# Autodesk Inventor assembly: Cockpit
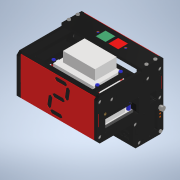
[picture p0: Inventor's stored thumbnail of the model, 180x180]
Saved by Autodesk Inventor 2020 (Build 240168000, 168)
## iProperties
Created: 2022-04-24
Part Number: Cockpit
Document SubType Name: Assembly
Designer: Masato Kubotera
Author: Masato Kubotera
## Documents named in this file (33)
- C:\Users\MasatoKubotera\Documents\Inventor\SUSTAINA-OP\UpperBody\Cockpit\Cockpit.iam
- C:\Users\MasatoKubotera\Documents\Inventor\SUSTAINA-OP\UpperBody\Cockpit\Cockpit_side_frame_MIR.ipt
- C:\Users\MasatoKubotera\Documents\Inventor\SUSTAINA-OP\UpperBody\Cockpit\Cockpit_battery_bottom_frame.ipt
- C:\Users\MasatoKubotera\Documents\Inventor\SUSTAINA-OP\UpperBody\Cockpit\Cockpit_battery_front_frame.ipt
- C:\Users\MasatoKubotera\Documents\Inventor\SUSTAINA-OP\UpperBody\Cockpit\Cockpit_front_frame.ipt
- C:\Users\MasatoKubotera\Documents\Inventor\SUSTAINA-OP\UpperBody\Cockpit\Cockpit_carrier_board_frame.ipt
- C:\Users\MasatoKubotera\Documents\Inventor\SUSTAINA-OP\UpperBody\Cockpit\Cockpit_back_frame.ipt
- C:\Users\MasatoKubotera\Documents\Inventor\SUSTAINA-OP\UpperBody\Cockpit\Cockpit_circuit_board_frame.ipt
- C:\Users\MasatoKubotera\Documents\Inventor\SUSTAINA-OP\UpperBody\Cockpit\Cockpit_battery_back_door.ipt
- C:\Users\MasatoKubotera\Documents\Inventor\SUSTAINA-OP\UpperBody\Cockpit\Cockpit_side_frame.ipt
- C:\Users\MasatoKubotera\Documents\Inventor\SUSTAINA-OP\ReadyMade\InsertNut\IRU-304S.ipt
- C:\Users\MasatoKubotera\Documents\Inventor\SUSTAINA-OP\ReadyMade\InsertNut\UD-43040.ipt
- C:\Users\MasatoKubotera\Documents\Inventor\SUSTAINA-OP\ReadyMade\Neodymium_magnet_Phi3_T3.ipt
- C:\Users\MasatoKubotera\Documents\Inventor\SUSTAINA-OP\UpperBody\Cockpit\Cockpit_front_frame_cloth.ipt
- C:\Users\MasatoKubotera\Documents\Inventor\SUSTAINA-OP\UpperBody\Cockpit\Cockpit_back_frame_cloth.ipt
- C:\Users\MasatoKubotera\Documents\Inventor\SUSTAINA-OP\ReadyMade\JetsonXavierNX_and_EN715.ipt
- C:\Users\MasatoKubotera\Documents\Inventor\SUSTAINA-OP\UpperBody\Cockpit\MainBoard.ipt
- C:\Users\MasatoKubotera\Documents\Inventor\SUSTAINA-OP\UpperBody\Cockpit\MainBoard_cover.ipt
- C:\Users\MasatoKubotera\Documents\Inventor\SUSTAINA-OP\ReadyMade\Battery\HP-G830C2800S3.ipt
- C:\Users\MasatoKubotera\Documents\Inventor\SUSTAINA-OP\ReadyMade\Screw\M3-6.ipt
- C:\Users\MasatoKubotera\Documents\Inventor\SUSTAINA-OP\ReadyMade\Screw\M3-10.ipt
- C:\Users\MasatoKubotera\Documents\Inventor\SUSTAINA-OP\ReadyMade\Screw\M3-8.ipt
- C:\Users\MasatoKubotera\Documents\Inventor\SUSTAINA-OP\UpperBody\Cockpit\Cockpit_top_frame.ipt
- C:\Users\MasatoKubotera\Documents\Inventor\SUSTAINA-OP\UpperBody\Cockpit\StartStopSwitch.ipt
- C:\Users\MasatoKubotera\Documents\Inventor\SUSTAINA-OP\ReadyMade\Spacer\ASL-313BE.ipt
- C:\Users\MasatoKubotera\Documents\Inventor\SUSTAINA-OP\ReadyMade\Spacer\BSL-306.5BE.ipt
- C:\Users\MasatoKubotera\Documents\Inventor\SUSTAINA-OP\UpperBody\Cockpit\ExpansionBoard.ipt
- C:\Users\MasatoKubotera\Documents\Inventor\SUSTAINA-OP\ReadyMade\Screw\M2_6-10.ipt
- C:\Users\MasatoKubotera\Documents\Inventor\SUSTAINA-OP\ReadyMade\Screw\SPNFL-BRN-M3-10.ipt
- C:\Users\MasatoKubotera\Documents\Inventor\SUSTAINA-OP\UpperBody\Cockpit\MainBoard_fan_plate.ipt
- C:\Users\MasatoKubotera\Documents\Inventor\SUSTAINA-OP\ReadyMade\YDM2507C12F.ipt
- C:\Users\MasatoKubotera\Documents\Inventor\SUSTAINA-OP\ReadyMade\Spacer\BRU-309S.ipt
- C:\Users\MasatoKubotera\Documents\Inventor\SUSTAINA-OP\ReadyMade\Screw\M2-6.ipt
## Components (121 placed, 32 different names)
1. MainBoard:1 — 挿入:63, 挿入:64, 挿入:65, 挿入:66, 挿入:95, 挿入:96, 挿入:148, 挿入:149
2. StartStopSwitch:1 — 挿入:103, 挿入:104, 挿入:105, 挿入:106
3. ExpansionBoard:1 — 挿入:123, 挿入:124, 挿入:125, 挿入:126, 挿入:127, 挿入:128, 挿入:129, 挿入:130
4. JetsonXavierNX_and_EN715:1 — 挿入:115, 挿入:116, 挿入:117, 挿入:118, 挿入:119, 挿入:120, 挿入:121, 挿入:122
5. M2-6:1 — 挿入:153
6. M2-6:2 — 挿入:152
7. Cockpit_side_frame_MIR:1 — 挿入:11, 挿入:12, 挿入:23, 挿入:24, 挿入:27, 挿入:28, 挿入:31, 挿入:32, 挿入:35, 挿入:36, 挿入:38, 挿入:40, 挿入:42, 挿入:46, 挿入:47, 挿入:48, 挿入:75, 挿入:77, 挿入:78, 挿入:79, 挿入:80, 挿入:81, 挿入:82, 挿入:134, 挿入:137
8. Cockpit_battery_bottom_frame:1 — 挿入:17, 挿入:18, 角度:2
9. Cockpit_battery_front_frame:1 — 挿入:19, 挿入:20, 角度:1
10. Cockpit_front_frame:1 — 挿入:1, 挿入:2, 挿入:3, フラッシュ:4, メイト:1
11. Cockpit_carrier_board_frame:1 — 挿入:5, 挿入:6, 挿入:7, 挿入:8, 挿入:89, 挿入:90, 挿入:91, 挿入:92, 挿入:111, 挿入:112, 挿入:113, 挿入:114
12. Cockpit_back_frame:1 — 挿入:13, 挿入:14, 挿入:15, 挿入:16, フラッシュ:7, メイト:2, 挿入:131, 挿入:132, 挿入:152, 挿入:153
13. Cockpit_circuit_board_frame:1 — メイト:3, メイト:4, フラッシュ:8, 挿入:55, 挿入:56, 挿入:57, 挿入:58
14. Cockpit_battery_back_door:1 — 挿入:41, 挿入:42, 挿入:49, 挿入:50, 挿入:51, 挿入:52, 挿入:53, 挿入:54, 角度:3
15. Cockpit_side_frame:1 — フラッシュ:1, フラッシュ:2, フラッシュ:3, 挿入:9, 挿入:10, 挿入:21, 挿入:22, 挿入:25, 挿入:26, 挿入:29, 挿入:30, 挿入:33, 挿入:34, 挿入:37, 挿入:39, 角度:1, 角度:2, 挿入:41, 挿入:43, 挿入:44, 挿入:45, フラッシュ:6, メイト:3, メイト:4, フラッシュ:8, 挿入:67, 挿入:68, 挿入:69, 挿入:70, 挿入:71, 挿入:72, 挿入:73, 挿入:74, 挿入:133, 角度:3, フラッシュ:5
16. Cockpit_front_frame_cloth:1 — フラッシュ:4, フラッシュ:5, メイト:1
17. Cockpit_back_frame_cloth:1 — フラッシュ:6, フラッシュ:7, メイト:2
18. Cockpit_top_frame:1 — 挿入:97, 挿入:98, 挿入:99, 挿入:100, 挿入:101, 挿入:102, 挿入:107, 挿入:108, 挿入:109, 挿入:110
19. MainBoard_cover:1 — 挿入:59, 挿入:60, 挿入:61, 挿入:62, 挿入:63, 挿入:64, 挿入:65, 挿入:66
20. MainBoard_fan_plate:1 — 挿入:138, 挿入:139, 挿入:140, 挿入:141, 挿入:146, 挿入:147, 挿入:150, 挿入:151
21. UD-43040:1 — 挿入:21
22. UD-43040:2 — 挿入:22, 挿入:83
23. UD-43040:3 — 挿入:23
24. UD-43040:4 — 挿入:24, 挿入:84
25. UD-43040:5 — 挿入:55, 挿入:59
26. UD-43040:6 — 挿入:56, 挿入:60
27. UD-43040:7 — 挿入:57, 挿入:61
28. UD-43040:8 — 挿入:58, 挿入:62
29. UD-43040:9 — 挿入:101, 挿入:103
30. UD-43040:10 — 挿入:102, 挿入:104
31. UD-43040:11 — 挿入:133, 挿入:135
32. UD-43040:12 — 挿入:134, 挿入:136
33. HP-G830C2800S3:1
34. ASL-313BE:1 — 挿入:115, 挿入:123
35. ASL-313BE:2 — 挿入:116, 挿入:124
36. ASL-313BE:3 — 挿入:117, 挿入:126
37. ASL-313BE:4 — 挿入:118, 挿入:125
38. BSL-306.5BE:1 — 挿入:111, 挿入:119
39. BSL-306.5BE:2 — 挿入:112, 挿入:120
40. BSL-306.5BE:3 — 挿入:113, 挿入:122
41. BSL-306.5BE:4 — 挿入:114, 挿入:121
42. BRU-309S:2 — 挿入:149, 挿入:151
43. BRU-309S:1 — 挿入:148, 挿入:150
44. IRU-304S:1 — 挿入:1, 挿入:25
45. IRU-304S:2 — 挿入:2, 挿入:26
46. IRU-304S:3 — 挿入:3, 挿入:27
47. IRU-304S:4 — 挿入:28
48. IRU-304S:5 — 挿入:5, 挿入:29
49. IRU-304S:6 — 挿入:6, 挿入:30
50. IRU-304S:7 — 挿入:7, 挿入:31
51. IRU-304S:8 — 挿入:8, 挿入:32
52. IRU-304S:9 — 挿入:9, 挿入:97
53. IRU-304S:10 — 挿入:10, 挿入:98
54. IRU-304S:11 — 挿入:11, 挿入:99
55. IRU-304S:12 — 挿入:12, 挿入:100
56. IRU-304S:13 — 挿入:13, 挿入:33
57. IRU-304S:14 — 挿入:14, 挿入:34
58. IRU-304S:15 — 挿入:15, 挿入:35
59. IRU-304S:16 — 挿入:16, 挿入:36
60. IRU-304S:17 — 挿入:17, 挿入:39
61. IRU-304S:18 — 挿入:18, 挿入:40
62. IRU-304S:19 — 挿入:19, 挿入:37
63. IRU-304S:20 — 挿入:20, 挿入:38
64. Neodymium_magnet_Phi3_T3:1 — 挿入:43
65. Neodymium_magnet_Phi3_T3:2 — 挿入:44
66. Neodymium_magnet_Phi3_T3:3 — 挿入:45
67. Neodymium_magnet_Phi3_T3:4 — 挿入:46
68. Neodymium_magnet_Phi3_T3:5 — 挿入:47
69. Neodymium_magnet_Phi3_T3:6 — 挿入:48
70. Neodymium_magnet_Phi3_T3:7 — 挿入:49
71. Neodymium_magnet_Phi3_T3:8 — 挿入:50
72. Neodymium_magnet_Phi3_T3:9 — 挿入:51
73. Neodymium_magnet_Phi3_T3:10 — 挿入:52
74. Neodymium_magnet_Phi3_T3:11 — 挿入:53
75. Neodymium_magnet_Phi3_T3:12 — 挿入:54
76. YDM2507C12F:1 — 挿入:138, 挿入:141, 挿入:142, 挿入:143
77. YDM2507C12F:2 — 挿入:139, 挿入:140, 挿入:144, 挿入:145
78. SPNFL-BRN-M3-10:2 — 挿入:136
79. SPNFL-BRN-M3-10:1 — 挿入:135
80. M2_6-10:1 — 挿入:131
81. M2_6-10:2 — 挿入:132
82. M3-6:1 — 挿入:67
83. M3-6:2 — 挿入:68
84. M3-6:3 — 挿入:69
85. M3-6:4 — 挿入:70
86. M3-6:5 — 挿入:71
87. M3-6:6 — 挿入:72
88. M3-6:7 — 挿入:73
89. M3-6:8 — 挿入:74
90. M3-6:9 — 挿入:75
91. M3-6:10 — 挿入:137
92. M3-6:11 — 挿入:77
93. M3-6:12 — 挿入:78
94. M3-6:13 — 挿入:79
95. M3-6:14 — 挿入:80
96. M3-6:15 — 挿入:81
97. M3-6:16 — 挿入:82
98. M3-6:17 — 挿入:105
99. M3-6:18 — 挿入:106
100. M3-6:19 — 挿入:127
101. M3-6:20 — 挿入:128
102. M3-6:21 — 挿入:129
103. M3-6:22 — 挿入:130
104. M3-6:23 — 挿入:146
105. M3-6:24 — 挿入:147
106. M3-8:1 — 挿入:89
107. M3-8:2 — 挿入:90
108. M3-8:3 — 挿入:91
109. M3-8:4 — 挿入:92
110. M3-8:7 — 挿入:95
111. M3-8:8 — 挿入:96
112. M3-8:9 — 挿入:107
113. M3-8:10 — 挿入:108
114. M3-8:11 — 挿入:109
115. M3-8:12 — 挿入:110
116. M3-10:1 — 挿入:83
117. M3-10:2 — 挿入:84
118. M3-10:3 — 挿入:142
119. M3-10:4 — 挿入:143
120. M3-10:5 — 挿入:144
121. M3-10:6 — 挿入:145
## Relationships (160: Insert 145, Flush 8, Mate 4, Angle 3)
- フラッシュ:1 [Flush]: Cockpit_side_frame:1
- フラッシュ:2 [Flush] (67.5 mm): Cockpit_side_frame:1
- フラッシュ:3 [Flush]: Cockpit_side_frame:1
- 挿入:1 [Insert]: Cockpit_front_frame:1 ↔ IRU-304S:1
- 挿入:2 [Insert]: Cockpit_front_frame:1 ↔ IRU-304S:2
- 挿入:3 [Insert]: Cockpit_front_frame:1 ↔ IRU-304S:3
- 挿入:5 [Insert]: Cockpit_carrier_board_frame:1 ↔ IRU-304S:5
- 挿入:6 [Insert]: Cockpit_carrier_board_frame:1 ↔ IRU-304S:6
- 挿入:7 [Insert]: Cockpit_carrier_board_frame:1 ↔ IRU-304S:7
- 挿入:8 [Insert]: Cockpit_carrier_board_frame:1 ↔ IRU-304S:8
- 挿入:9 [Insert]: Cockpit_side_frame:1 ↔ IRU-304S:9
- 挿入:10 [Insert]: Cockpit_side_frame:1 ↔ IRU-304S:10
- 挿入:11 [Insert]: Cockpit_side_frame_MIR:1 ↔ IRU-304S:11
- 挿入:12 [Insert]: Cockpit_side_frame_MIR:1 ↔ IRU-304S:12
- 挿入:13 [Insert]: Cockpit_back_frame:1 ↔ IRU-304S:13
- 挿入:14 [Insert]: Cockpit_back_frame:1 ↔ IRU-304S:14
- 挿入:15 [Insert]: Cockpit_back_frame:1 ↔ IRU-304S:15
- 挿入:16 [Insert]: Cockpit_back_frame:1 ↔ IRU-304S:16
- 挿入:17 [Insert]: Cockpit_battery_bottom_frame:1 ↔ IRU-304S:17
- 挿入:18 [Insert]: Cockpit_battery_bottom_frame:1 ↔ IRU-304S:18
- 挿入:19 [Insert]: Cockpit_battery_front_frame:1 ↔ IRU-304S:19
- 挿入:20 [Insert]: Cockpit_battery_front_frame:1 ↔ IRU-304S:20
- 挿入:21 [Insert]: Cockpit_side_frame:1 ↔ UD-43040:1
- 挿入:22 [Insert]: Cockpit_side_frame:1 ↔ UD-43040:2
- 挿入:23 [Insert]: Cockpit_side_frame_MIR:1 ↔ UD-43040:3
- 挿入:24 [Insert]: Cockpit_side_frame_MIR:1 ↔ UD-43040:4
- 挿入:25 [Insert]: Cockpit_side_frame:1 ↔ IRU-304S:1
- 挿入:26 [Insert]: Cockpit_side_frame:1 ↔ IRU-304S:2
- 挿入:27 [Insert]: Cockpit_side_frame_MIR:1 ↔ IRU-304S:3
- 挿入:28 [Insert]: Cockpit_side_frame_MIR:1 ↔ IRU-304S:4
- 挿入:29 [Insert]: Cockpit_side_frame:1 ↔ IRU-304S:5
- 挿入:30 [Insert]: Cockpit_side_frame:1 ↔ IRU-304S:6
- 挿入:31 [Insert]: Cockpit_side_frame_MIR:1 ↔ IRU-304S:7
- 挿入:32 [Insert]: Cockpit_side_frame_MIR:1 ↔ IRU-304S:8
- 挿入:33 [Insert]: Cockpit_side_frame:1 ↔ IRU-304S:13
- 挿入:34 [Insert]: Cockpit_side_frame:1 ↔ IRU-304S:14
- 挿入:35 [Insert]: Cockpit_side_frame_MIR:1 ↔ IRU-304S:15
- 挿入:36 [Insert]: Cockpit_side_frame_MIR:1 ↔ IRU-304S:16
- 挿入:37 [Insert]: Cockpit_side_frame:1 ↔ IRU-304S:19
- 挿入:38 [Insert]: Cockpit_side_frame_MIR:1 ↔ IRU-304S:20
- 挿入:39 [Insert]: Cockpit_side_frame:1 ↔ IRU-304S:17
- 挿入:40 [Insert]: Cockpit_side_frame_MIR:1 ↔ IRU-304S:18
- 角度:1 [Angle] (0 deg): Cockpit_battery_front_frame:1 ↔ Cockpit_side_frame:1
- 角度:2 [Angle] (0 deg): Cockpit_battery_bottom_frame:1 ↔ Cockpit_side_frame:1
- 挿入:41 [Insert]: Cockpit_battery_back_door:1 ↔ Cockpit_side_frame:1
- 挿入:42 [Insert]: Cockpit_side_frame_MIR:1 ↔ Cockpit_battery_back_door:1
- 挿入:43 [Insert]: Cockpit_side_frame:1 ↔ Neodymium_magnet_Phi3_T3:1
- 挿入:44 [Insert]: Cockpit_side_frame:1 ↔ Neodymium_magnet_Phi3_T3:2
- 挿入:45 [Insert]: Cockpit_side_frame:1 ↔ Neodymium_magnet_Phi3_T3:3
- 挿入:46 [Insert]: Cockpit_side_frame_MIR:1 ↔ Neodymium_magnet_Phi3_T3:4
- 挿入:47 [Insert]: Cockpit_side_frame_MIR:1 ↔ Neodymium_magnet_Phi3_T3:5
- 挿入:48 [Insert]: Cockpit_side_frame_MIR:1 ↔ Neodymium_magnet_Phi3_T3:6
- 挿入:49 [Insert]: Cockpit_battery_back_door:1 ↔ Neodymium_magnet_Phi3_T3:7
- 挿入:50 [Insert]: Cockpit_battery_back_door:1 ↔ Neodymium_magnet_Phi3_T3:8
- 挿入:51 [Insert]: Cockpit_battery_back_door:1 ↔ Neodymium_magnet_Phi3_T3:9
- 挿入:52 [Insert]: Cockpit_battery_back_door:1 ↔ Neodymium_magnet_Phi3_T3:10
- 挿入:53 [Insert]: Cockpit_battery_back_door:1 ↔ Neodymium_magnet_Phi3_T3:11
- 挿入:54 [Insert]: Cockpit_battery_back_door:1 ↔ Neodymium_magnet_Phi3_T3:12
- フラッシュ:4 [Flush]: Cockpit_front_frame:1 ↔ Cockpit_front_frame_cloth:1
- フラッシュ:5 [Flush]: Cockpit_side_frame:1 ↔ Cockpit_front_frame_cloth:1
- メイト:1 [Mate]: Cockpit_front_frame:1 ↔ Cockpit_front_frame_cloth:1
- フラッシュ:6 [Flush]: Cockpit_side_frame:1 ↔ Cockpit_back_frame_cloth:1
- フラッシュ:7 [Flush]: Cockpit_back_frame:1 ↔ Cockpit_back_frame_cloth:1
- メイト:2 [Mate]: Cockpit_back_frame:1 ↔ Cockpit_back_frame_cloth:1
- メイト:3 [Mate] (0.05 mm): Cockpit_circuit_board_frame:1 ↔ Cockpit_side_frame:1
- メイト:4 [Mate] (0.05 mm): Cockpit_circuit_board_frame:1 ↔ Cockpit_side_frame:1
- フラッシュ:8 [Flush]: Cockpit_circuit_board_frame:1 ↔ Cockpit_side_frame:1
- 挿入:55 [Insert]: Cockpit_circuit_board_frame:1 ↔ UD-43040:5
- 挿入:56 [Insert]: Cockpit_circuit_board_frame:1 ↔ UD-43040:6
- 挿入:57 [Insert]: Cockpit_circuit_board_frame:1 ↔ UD-43040:7
- 挿入:58 [Insert]: Cockpit_circuit_board_frame:1 ↔ UD-43040:8
- 挿入:59 [Insert]: MainBoard_cover:1 ↔ UD-43040:5
- 挿入:60 [Insert]: MainBoard_cover:1 ↔ UD-43040:6
- 挿入:61 [Insert]: MainBoard_cover:1 ↔ UD-43040:7
- 挿入:62 [Insert]: MainBoard_cover:1 ↔ UD-43040:8
- 挿入:63 [Insert]: MainBoard:1 ↔ MainBoard_cover:1
- 挿入:64 [Insert]: MainBoard:1 ↔ MainBoard_cover:1
- 挿入:65 [Insert]: MainBoard:1 ↔ MainBoard_cover:1
- 挿入:66 [Insert]: MainBoard:1 ↔ MainBoard_cover:1
- 挿入:67 [Insert]: Cockpit_side_frame:1 ↔ M3-6:1
- 挿入:68 [Insert]: Cockpit_side_frame:1 ↔ M3-6:2
- 挿入:69 [Insert]: Cockpit_side_frame:1 ↔ M3-6:3
- 挿入:70 [Insert]: Cockpit_side_frame:1 ↔ M3-6:4
- 挿入:71 [Insert]: Cockpit_side_frame:1 ↔ M3-6:5
- 挿入:72 [Insert]: Cockpit_side_frame:1 ↔ M3-6:6
- 挿入:73 [Insert]: Cockpit_side_frame:1 ↔ M3-6:7
- 挿入:74 [Insert]: Cockpit_side_frame:1 ↔ M3-6:8
- 挿入:75 [Insert]: Cockpit_side_frame_MIR:1 ↔ M3-6:9
- 挿入:77 [Insert]: Cockpit_side_frame_MIR:1 ↔ M3-6:11
- 挿入:78 [Insert]: Cockpit_side_frame_MIR:1 ↔ M3-6:12
- 挿入:79 [Insert]: Cockpit_side_frame_MIR:1 ↔ M3-6:13
- 挿入:80 [Insert]: Cockpit_side_frame_MIR:1 ↔ M3-6:14
- 挿入:81 [Insert]: Cockpit_side_frame_MIR:1 ↔ M3-6:15
- 挿入:82 [Insert]: Cockpit_side_frame_MIR:1 ↔ M3-6:16
- 挿入:83 [Insert]: UD-43040:2 ↔ M3-10:1
- 挿入:84 [Insert]: UD-43040:4 ↔ M3-10:2
- 挿入:89 [Insert]: Cockpit_carrier_board_frame:1 ↔ M3-8:1
- 挿入:90 [Insert]: Cockpit_carrier_board_frame:1 ↔ M3-8:2
- 挿入:91 [Insert]: Cockpit_carrier_board_frame:1 ↔ M3-8:3
- 挿入:92 [Insert]: Cockpit_carrier_board_frame:1 ↔ M3-8:4
- 挿入:95 [Insert]: MainBoard:1 ↔ M3-8:7
- 挿入:96 [Insert]: MainBoard:1 ↔ M3-8:8
- 挿入:97 [Insert]: Cockpit_top_frame:1 ↔ IRU-304S:9
- 挿入:98 [Insert]: Cockpit_top_frame:1 ↔ IRU-304S:10
- 挿入:99 [Insert]: Cockpit_top_frame:1 ↔ IRU-304S:11
- 挿入:100 [Insert]: Cockpit_top_frame:1 ↔ IRU-304S:12
- 挿入:101 [Insert]: Cockpit_top_frame:1 ↔ UD-43040:9
- 挿入:102 [Insert]: Cockpit_top_frame:1 ↔ UD-43040:10
- 挿入:103 [Insert]: StartStopSwitch:1 ↔ UD-43040:9
- 挿入:104 [Insert]: StartStopSwitch:1 ↔ UD-43040:10
- 挿入:105 [Insert]: StartStopSwitch:1 ↔ M3-6:17
- 挿入:106 [Insert]: StartStopSwitch:1 ↔ M3-6:18
- 挿入:107 [Insert]: Cockpit_top_frame:1 ↔ M3-8:9
- 挿入:108 [Insert]: Cockpit_top_frame:1 ↔ M3-8:10
- 挿入:109 [Insert]: Cockpit_top_frame:1 ↔ M3-8:11
- 挿入:110 [Insert]: Cockpit_top_frame:1 ↔ M3-8:12
- 挿入:111 [Insert]: Cockpit_carrier_board_frame:1 ↔ BSL-306.5BE:1
- 挿入:112 [Insert]: Cockpit_carrier_board_frame:1 ↔ BSL-306.5BE:2
- 挿入:113 [Insert]: Cockpit_carrier_board_frame:1 ↔ BSL-306.5BE:3
- 挿入:114 [Insert]: Cockpit_carrier_board_frame:1 ↔ BSL-306.5BE:4
- 挿入:115 [Insert]: JetsonXavierNX_and_EN715:1 ↔ ASL-313BE:1
- 挿入:116 [Insert]: JetsonXavierNX_and_EN715:1 ↔ ASL-313BE:2
- 挿入:117 [Insert]: JetsonXavierNX_and_EN715:1 ↔ ASL-313BE:3
- 挿入:118 [Insert]: JetsonXavierNX_and_EN715:1 ↔ ASL-313BE:4
- 挿入:119 [Insert]: JetsonXavierNX_and_EN715:1 ↔ BSL-306.5BE:1
- 挿入:120 [Insert]: JetsonXavierNX_and_EN715:1 ↔ BSL-306.5BE:2
- 挿入:121 [Insert]: JetsonXavierNX_and_EN715:1 ↔ BSL-306.5BE:4
- 挿入:122 [Insert]: JetsonXavierNX_and_EN715:1 ↔ BSL-306.5BE:3
- 挿入:123 [Insert]: ExpansionBoard:1 ↔ ASL-313BE:1
- 挿入:124 [Insert]: ExpansionBoard:1 ↔ ASL-313BE:2
- 挿入:125 [Insert]: ExpansionBoard:1 ↔ ASL-313BE:4
- 挿入:126 [Insert]: ExpansionBoard:1 ↔ ASL-313BE:3
- 挿入:127 [Insert]: ExpansionBoard:1 ↔ M3-6:19
- 挿入:128 [Insert]: ExpansionBoard:1 ↔ M3-6:20
- 挿入:129 [Insert]: ExpansionBoard:1 ↔ M3-6:21
- 挿入:130 [Insert]: ExpansionBoard:1 ↔ M3-6:22
- 挿入:131 [Insert]: Cockpit_back_frame:1 ↔ M2_6-10:1
- 挿入:132 [Insert]: Cockpit_back_frame:1 ↔ M2_6-10:2
- 挿入:133 [Insert]: Cockpit_side_frame:1 ↔ UD-43040:11
- 挿入:134 [Insert]: Cockpit_side_frame_MIR:1 ↔ UD-43040:12
- 挿入:135 [Insert]: UD-43040:11 ↔ SPNFL-BRN-M3-10:1
- 挿入:136 [Insert]: UD-43040:12 ↔ SPNFL-BRN-M3-10:2
- 角度:3 [Angle] (0 deg): Cockpit_battery_back_door:1 ↔ Cockpit_side_frame:1
- 挿入:137 [Insert]: Cockpit_side_frame_MIR:1 ↔ M3-6:10
- 挿入:138 [Insert]: MainBoard_fan_plate:1 ↔ YDM2507C12F:1
- 挿入:139 [Insert]: MainBoard_fan_plate:1 ↔ YDM2507C12F:2
- 挿入:140 [Insert]: MainBoard_fan_plate:1 ↔ YDM2507C12F:2
- 挿入:141 [Insert]: MainBoard_fan_plate:1 ↔ YDM2507C12F:1
- 挿入:142 [Insert]: YDM2507C12F:1 ↔ M3-10:3
- 挿入:143 [Insert]: YDM2507C12F:1 ↔ M3-10:4
- 挿入:144 [Insert]: YDM2507C12F:2 ↔ M3-10:5
- 挿入:145 [Insert]: YDM2507C12F:2 ↔ M3-10:6
- 挿入:146 [Insert]: MainBoard_fan_plate:1 ↔ M3-6:23
- 挿入:147 [Insert]: MainBoard_fan_plate:1 ↔ M3-6:24
- 挿入:148 [Insert]: MainBoard:1 ↔ BRU-309S:1
- 挿入:149 [Insert]: MainBoard:1 ↔ BRU-309S:2
- 挿入:150 [Insert]: MainBoard_fan_plate:1 ↔ BRU-309S:1
- 挿入:151 [Insert]: MainBoard_fan_plate:1 ↔ BRU-309S:2
- 挿入:152 [Insert]: M2-6:2 ↔ Cockpit_back_frame:1
- 挿入:153 [Insert]: M2-6:1 ↔ Cockpit_back_frame:1
